# Autodesk Inventor assembly: FE-100 Side Wall
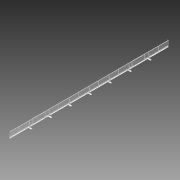
[picture p0: Inventor's stored thumbnail of the model, 180x180]
Saved by Autodesk Inventor 2021 (Build 250183000, 183)
## iProperties
Created: 2021-01-11
Part Number: FE-100 Side Wall
Document SubType Name: Assembly
## Documents named in this file (8)
- D:\FIRST\Design\FRC Fields\Generic Field Base\FE-100 Side Wall\FE-100 Side Wall.iam
- D:\FIRST\Design\FRC Fields\Generic Field Base\FE-100 Side Wall\FE-110 Main Section\FE-100 Main Section.iam
- D:\FIRST\Design\FRC Fields\Generic Field Base\FE-100 Side Wall\FE-110 Main Section\FE-100 Main Section No Insert.iam
- D:\FIRST\Design\FRC Fields\Generic Field Base\FE-100 Side Wall\FE-130 End-Cap\FE-130 End-Cap.iam
- D:\FIRST\Design\FRC Fields\Generic Field Base\FE-100 Side Wall\FE-120 Door Section\FE-120 Door Section.iam
- D:\FIRST\Design\FRC Fields\Generic Field Base\FE-100 Side Wall\FE-100-001 Main Panel.ipt
- D:\FIRST\Design\FRC Fields\Generic Field Base\FE-100 Side Wall\FE-100-002 Secondary Panel.ipt
- D:\FIRST\Design\FRC Fields\Generic Field Base\FE-100 Side Wall\FE-100-003 End Panel.ipt
## Components (19 placed, 7 different names)
1. FE-100 Main Section:5 [sub-assembly] — Mate:3, Mate:4, Mate:10, Mate:11, Mate:12, Mate:13, Mate:18, Tangent:2
2. FE-100 Main Section No Insert:1 [sub-assembly] — Mate:5, Mate:6, Mate:7, Mate:8, Mate:9, Flush:2, Mate:15, Tangent:3
3. FE-130 End-Cap:1 [sub-assembly] — Mate:7, Mate:8, Mate:9, Symmetry:1, Flush:11, Mate:23
4. FE-130 End-Cap:2 [sub-assembly] — Mate:10, Mate:11, Mate:12, Symmetry:1, Flush:10, Mate:22
5. FE-120 Door Section:1 [sub-assembly] — Mate:13, Flush:1, Mate:16, Mate:18, Flush:9
6. FE-120 Door Section:2 [sub-assembly] — Mate:14, Flush:2, Mate:15, Mate:19
7. FE-100-002 Secondary Panel:1 — Flush:5, Flush:6, Flush:9, Mate:20
8. FE-100-002 Secondary Panel:2 — Flush:5, Flush:6, Tangent:2, Flush:10, Flush:12, Flush:13
9. FE-100-002 Secondary Panel:3 — Flush:4, Flush:7, Flush:8, Mate:21
10. FE-100-002 Secondary Panel:4 — Flush:4, Flush:7, Tangent:3, Flush:11, Flush:14, Flush:15
11. FE-100-003 End Panel:2 — Mate:23, Flush:14, Flush:15
12. FE-100-003 End Panel:3 — Mate:22, Flush:12, Flush:13
13. FE-100 Main Section:1 [sub-assembly] — Mate:1, Mate:2, Mate:3, Mate:4, Flush:1, Mate:16, Tangent:1, Mate:17
14. FE-100 Main Section:2 [sub-assembly] — Flush:3
15. FE-100 Main Section:3 [sub-assembly] — Flush:8
16. FE-100 Main Section:4 [sub-assembly] — Mate:5, Mate:6, Mate:14, Mate:19
17. FE-100-001 Main Panel:1 — Tangent:1, Flush:3, Mate:17, Mate:20
18. FE-100-001 Main Panel:2
19. FE-100-001 Main Panel:3 — Mate:21
## Component patterns: (4 elements, first: FE-100 Main Section:1), (3 elements, first: FE-100-001 Main Panel:1)
## Relationships (42: Mate 23, Flush 15, Tangent 3, Symmetry 1)
- Mate:1: FE-100 Main Section:1
- Mate:2: FE-100 Main Section:1
- Mate:3: FE-100 Main Section:5 ↔ FE-100 Main Section:1
- Mate:4: FE-100 Main Section:5 ↔ FE-100 Main Section:1
- Mate:5: FE-100 Main Section No Insert:1 ↔ FE-100 Main Section:4
- Mate:6: FE-100 Main Section No Insert:1 ↔ FE-100 Main Section:4
- Mate:7: FE-100 Main Section No Insert:1 ↔ FE-130 End-Cap:1
- Mate:8: FE-100 Main Section No Insert:1 ↔ FE-130 End-Cap:1
- Mate:9: FE-100 Main Section No Insert:1 ↔ FE-130 End-Cap:1
- Mate:10: FE-100 Main Section:5 ↔ FE-130 End-Cap:2
- Mate:11: FE-100 Main Section:5 ↔ FE-130 End-Cap:2
- Mate:12: FE-100 Main Section:5 ↔ FE-130 End-Cap:2
- Symmetry:1: FE-130 End-Cap:1 ↔ FE-130 End-Cap:2
- Mate:13: FE-100 Main Section:5 ↔ FE-120 Door Section:1
- Mate:14: FE-120 Door Section:2 ↔ FE-100 Main Section:4
- Flush:1: FE-120 Door Section:1 ↔ FE-100 Main Section:1
- Flush:2: FE-100 Main Section No Insert:1 ↔ FE-120 Door Section:2
- Mate:15: FE-100 Main Section No Insert:1 ↔ FE-120 Door Section:2
- Mate:16: FE-120 Door Section:1 ↔ FE-100 Main Section:1
- Tangent:1 (4.826 mm): FE-100 Main Section:1 ↔ FE-100-001 Main Panel:1
- Flush:3: FE-100 Main Section:2 ↔ FE-100-001 Main Panel:1
- Mate:17: FE-100 Main Section:1 ↔ FE-100-001 Main Panel:1
- Mate:18: FE-100 Main Section:5 ↔ FE-120 Door Section:1
- Mate:19: FE-120 Door Section:2 ↔ FE-100 Main Section:4
- Flush:4: FE-100-002 Secondary Panel:3 ↔ FE-100-002 Secondary Panel:4
- Flush:5: FE-100-002 Secondary Panel:1 ↔ FE-100-002 Secondary Panel:2
- Flush:6: FE-100-002 Secondary Panel:1 ↔ FE-100-002 Secondary Panel:2
- Flush:7: FE-100-002 Secondary Panel:3 ↔ FE-100-002 Secondary Panel:4
- Flush:8: FE-100-002 Secondary Panel:3 ↔ FE-100 Main Section:3
- Flush:9: FE-120 Door Section:1 ↔ FE-100-002 Secondary Panel:1
- Tangent:2 (4.826 mm): FE-100 Main Section:5 ↔ FE-100-002 Secondary Panel:2
- Tangent:3 (4.826 mm): FE-100 Main Section No Insert:1 ↔ FE-100-002 Secondary Panel:4
- Flush:10 (931.926 mm): FE-130 End-Cap:2 ↔ FE-100-002 Secondary Panel:2
- Flush:11 (-931.926 mm): FE-130 End-Cap:1 ↔ FE-100-002 Secondary Panel:4
- Mate:20 (4.826 mm): FE-100-002 Secondary Panel:1 ↔ FE-100-001 Main Panel:1
- Mate:21 (4.826 mm): FE-100-002 Secondary Panel:3 ↔ FE-100-001 Main Panel:3
- Mate:22 (4.826 mm): FE-130 End-Cap:2 ↔ FE-100-003 End Panel:3
- Flush:12: FE-100-002 Secondary Panel:2 ↔ FE-100-003 End Panel:3
- Flush:13: FE-100-002 Secondary Panel:2 ↔ FE-100-003 End Panel:3
- Mate:23 (4.826 mm): FE-130 End-Cap:1 ↔ FE-100-003 End Panel:2
- Flush:14: FE-100-002 Secondary Panel:4 ↔ FE-100-003 End Panel:2
- Flush:15: FE-100-002 Secondary Panel:4 ↔ FE-100-003 End Panel:2
